# Autodesk Inventor assembly: Wheel
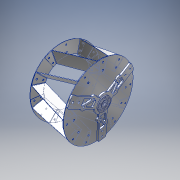
[picture p0: Inventor's stored thumbnail of the model, 180x180]
Saved by Autodesk Inventor 2019 (Build 230136000, 136)
## iProperties
Created: 2017-04-20
Part Number: Wheel
Document SubType Name: Assembly
Designer: Adhikara
Mass: 1032.4 g
Surface Area: 4830.7 cm^2
Volume: 382.369 cm^3
Density: 2.7 g/cm^3
Author: Adhikara
## Documents named in this file (6)
- I:\CAD\Julie\Wheel.iam
- I:\CAD\Julie\Wall.ipt
- I:\CAD\Julie\Edge.ipt
- I:\CAD\Julie\Rim.ipt
- I:\CAD\Julie\Key Hub.ipt
- C:\Users\Adhik\Documents\CAD\AR10\AR10\Doubler.ipt
## Components (12 placed, 5 different names)
1. Wall:1 — Mate:1, Mate:2, Mate:3, Mate:4, Mate:5, Mate:6, Flush:1
2. Rim:1 — Mate:7, Mate:8
3. Key Hub:1 — Mate:9, Mate:10, Mate:11
4. Edge:2 — Mate:4, Mate:5, Mate:6, Mate:8
5. Edge:1 — Mate:1, Mate:2, Mate:3
6. Edge:3
7. Edge:4
8. Edge:5
9. Edge:6
10. Doubler:1 — Flush:1
11. Doubler:2
12. Doubler:3 — Mate:10, Mate:11
## Component patterns: (3 elements, first: Edge:2 + Edge:1), (3 elements, first: Doubler:1)
## Relationships (12: Mate 11, Flush 1)
- Mate:1: Wall:1 ↔ Edge:1
- Mate:2: Wall:1 ↔ Edge:1
- Mate:3: Wall:1 ↔ Edge:1
- Mate:4: Wall:1 ↔ Edge:2
- Mate:5: Wall:1 ↔ Edge:2
- Mate:6: Wall:1 ↔ Edge:2
- Mate:7: Rim:1
- Mate:8: Rim:1 ↔ Edge:2
- Mate:9: Key Hub:1
- Flush:1: Wall:1 ↔ Doubler:1
- Mate:10: Key Hub:1 ↔ Doubler:3
- Mate:11: Key Hub:1 ↔ Doubler:3
